# Autodesk Inventor assembly: ASM_Coupler_Bearing_ID
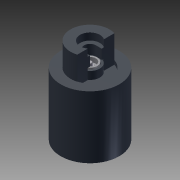
[picture p0: Inventor's stored thumbnail of the model, 180x180]
Saved by Autodesk Inventor 2011 SP2 (Build 150309200, 309)
## iProperties
Created: 2012-02-15
Part Number: ASM_Coupler_Bearing_ID
Document SubType Name: Assembly
Designer: sungwook
Author: sungwook
## Documents named in this file (6)
- C:\Users\sungwook\Documents\Inventor\Micron20\Assembly\ASM_Coupler_Bearing_ID.iam
- C:\Users\sungwook\Documents\Inventor\Micron20\Parts\Jigs\Bearing_ID_Asm_Base.ipt
- C:\Users\sungwook\Documents\Inventor\Micron20\Parts\Motor Units\MU_Motor_Coupling_3.ipt
- C:\Users\sungwook\Documents\Inventor\Micron20\Parts\Motor Units\MU_Motor_Thread.ipt
- C:\Users\sungwook\Documents\Inventor\Micron20\Parts\Jigs\Bearing_ID_Asm_Holder.ipt
- C:\Users\sungwook\Documents\Inventor\Micron20\Parts\Motor Units\MU_Bearing_Retainer.ipt
## Components (5 placed, 5 different names)
1. Bearing_ID_Asm_Base:1 — Mate:3, Mate:4, Mate:5, Mate:8
2. MU_Motor_Coupling_3:1 — Mate:1, Mate:2, Mate:3, Mate:4, Mate:6, Mate:7
3. MU_Motor_Thread:1 — Mate:1, Mate:2
4. Bearing_ID_Asm_Holder:1 — Mate:5, Mate:8, Flush:1
5. MU_Bearing_Retainer:1 — Mate:6, Mate:7
## Relationships (9: Mate 8, Flush 1)
- Mate:1: MU_Motor_Coupling_3:1 ↔ MU_Motor_Thread:1
- Mate:2: MU_Motor_Coupling_3:1 ↔ MU_Motor_Thread:1
- Mate:3: Bearing_ID_Asm_Base:1 ↔ MU_Motor_Coupling_3:1
- Mate:4: Bearing_ID_Asm_Base:1 ↔ MU_Motor_Coupling_3:1
- Mate:5: Bearing_ID_Asm_Base:1 ↔ Bearing_ID_Asm_Holder:1
- Mate:6: MU_Motor_Coupling_3:1 ↔ MU_Bearing_Retainer:1
- Mate:7: MU_Motor_Coupling_3:1 ↔ MU_Bearing_Retainer:1
- Mate:8: Bearing_ID_Asm_Base:1 ↔ Bearing_ID_Asm_Holder:1
- Flush:1: Bearing_ID_Asm_Holder:1
